# Autodesk Inventor assembly: A2017_T4_02
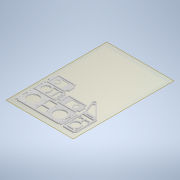
[picture p0: Inventor's stored thumbnail of the model, 180x180]
Saved by Autodesk Inventor 2020 (Build 240168000, 168)
## iProperties
Created: 2021-08-27
Part Number: A2017_T4_02
Document SubType Name: Assembly
Designer: Masato
Author: Masato
## Documents named in this file (6)
- C:\Inventor\SUSTAINA-OP\Cam\A2017_T4_02.iam
- C:\Inventor\SUSTAINA-OP\Cam\DisposableBoard.ipt
- C:\Inventor\SUSTAINA-OP\UpperBody\Trunk\Trunk_neck_frame.ipt
- C:\Inventor\SUSTAINA-OP\UpperBody\Trunk\Trunk_shoulder_frame.ipt
- C:\Inventor\SUSTAINA-OP\UpperBody\Trunk\Trunk_waisit_frame.ipt
- C:\Inventor\SUSTAINA-OP\UpperBody\Trunk\Trunk_servo_bottom_frame.ipt
## Components (6 placed, 5 different names)
1. DisposableBoard:1 — メイト:2, メイト:1, フラッシュ:1, フラッシュ:2, フラッシュ:3, フラッシュ:5, メイト:17, メイト:21
2. Trunk_neck_frame:1 — メイト:6, フラッシュ:6, メイト:16, メイト:19, メイト:20
3. Trunk_shoulder_frame:1 — メイト:9, フラッシュ:4, メイト:15
4. Trunk_waisit_frame:1 — フラッシュ:3, フラッシュ:4, フラッシュ:5, フラッシュ:6, メイト:15, メイト:16, メイト:18, フラッシュ:7, メイト:21
5. Trunk_servo_bottom_frame:2 — メイト:14, メイト:20, フラッシュ:7
6. Trunk_servo_bottom_frame:1 — メイト:17, メイト:18, メイト:19
## Relationships (19: Mate 12, Flush 7)
- メイト:2 [Mate]: DisposableBoard:1
- メイト:1 [Mate]: DisposableBoard:1
- フラッシュ:1 [Flush]: DisposableBoard:1
- フラッシュ:2 [Flush]: DisposableBoard:1
- メイト:6 [Mate]: Trunk_neck_frame:1
- メイト:9 [Mate]: Trunk_shoulder_frame:1
- メイト:14 [Mate]: Trunk_servo_bottom_frame:2
- フラッシュ:3 [Flush] (2 mm): DisposableBoard:1 ↔ Trunk_waisit_frame:1
- フラッシュ:4 [Flush]: Trunk_shoulder_frame:1 ↔ Trunk_waisit_frame:1
- フラッシュ:5 [Flush] (1.75 mm): DisposableBoard:1 ↔ Trunk_waisit_frame:1
- フラッシュ:6 [Flush]: Trunk_neck_frame:1 ↔ Trunk_waisit_frame:1
- メイト:15 [Mate] (2.5 mm): Trunk_shoulder_frame:1 ↔ Trunk_waisit_frame:1
- メイト:16 [Mate] (2.5 mm): Trunk_neck_frame:1 ↔ Trunk_waisit_frame:1
- メイト:17 [Mate]: DisposableBoard:1 ↔ Trunk_servo_bottom_frame:1
- メイト:18 [Mate] (2.5 mm): Trunk_waisit_frame:1 ↔ Trunk_servo_bottom_frame:1
- メイト:19 [Mate] (2.5 mm): Trunk_neck_frame:1 ↔ Trunk_servo_bottom_frame:1
- メイト:20 [Mate] (2.5 mm): Trunk_neck_frame:1 ↔ Trunk_servo_bottom_frame:2
- フラッシュ:7 [Flush]: Trunk_waisit_frame:1 ↔ Trunk_servo_bottom_frame:2
- メイト:21 [Mate]: DisposableBoard:1 ↔ Trunk_waisit_frame:1
